# Autodesk Inventor assembly: AlternateServoMount
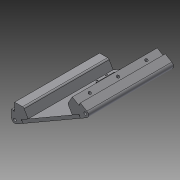
[picture p0: Inventor's stored thumbnail of the model, 180x180]
Saved by Autodesk Inventor 2014 SP1 (Build 180222100, 222)
## iProperties
Created: 2014-11-10
Part Number: AlternateServoMount
Document SubType Name: Assembly
Designer: rawrdong
Author: rawrdong
## Documents named in this file (3)
- C:\Users\rawrdong\Documents\GitHub\FlippityFlappity\CAD_HW\AlternateServoMount.iam
- C:\Users\rawrdong\Documents\GitHub\FlippityFlappity\CAD_HW\ServoHousing_alternateLaser.ipt
- C:\Users\rawrdong\Documents\GitHub\FlippityFlappity\CAD_HW\ServoPlate1.ipt
## Components (3 placed, 2 different names)
1. ServoHousing_alternateLaser:1 — Mate:1, Mate:2, Mate:3
2. ServoPlate1:1 — Mate:1, Mate:2, Mate:3, Mate:4, Mate:5, Mate:6
3. ServoHousing_alternateLaser:2 — Mate:4, Mate:5, Mate:6
## Relationships (6: Mate 6)
- Mate:1: ServoHousing_alternateLaser:1 ↔ ServoPlate1:1
- Mate:2: ServoHousing_alternateLaser:1 ↔ ServoPlate1:1
- Mate:3: ServoHousing_alternateLaser:1 ↔ ServoPlate1:1
- Mate:4: ServoPlate1:1 ↔ ServoHousing_alternateLaser:2
- Mate:5: ServoPlate1:1 ↔ ServoHousing_alternateLaser:2
- Mate:6: ServoPlate1:1 ↔ ServoHousing_alternateLaser:2
